# Autodesk Inventor assembly: 39079
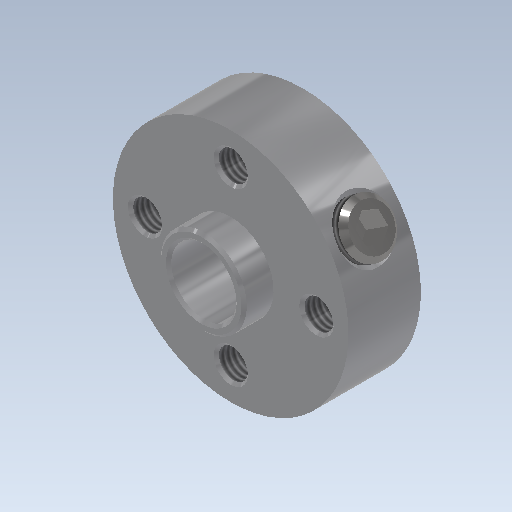
[picture p0: Inventor's stored thumbnail of the model, 512x512]
Saved by Autodesk Inventor 2020 (Build 240168000, 168)
## iProperties
Created: 2017-01-02
Part Number: 39079
Document SubType Name: Assembly
Designer: Autodesk Inc.
Catalog Web Link: http://www.tetrixrobotics.com/TETRIX_Motor_Shaft_Hubs
Vendor: Tetrix
Category: Wheel Hardware
Company: Autodesk Inc.
Author: Autodesk Inc.
## Documents named in this file (3)
- D:\Documents\GitHub\AO_Robotics\CAD\Parts Kits\FTC Tetrix KOP Organized (7-24-19)\Axle Hardware\Tetrix_39079.iam
- D:\Documents\GitHub\AO_Robotics\CAD\Parts Kits\FTC Tetrix KOP Organized (7-24-19)\Axle Hardware\Assembly Components\Tetrix_39079_Collar.ipt
- D:\Documents\GitHub\AO_Robotics\CAD\Parts Kits\FTC Tetrix KOP Organized (7-24-19)\Axle Hardware\Assembly Components\Tetrix_39079_Screw.ipt
## Components (2 placed, 2 different names)
1. Tetrix_39079_Collar:1 — Mate:1
2. Tetrix_39079_Screw:1 — Mate:1
## Relationships (1: Mate 1)
- Mate:1: Tetrix_39079_Collar:1 ↔ Tetrix_39079_Screw:1
